# Autodesk Inventor assembly: Servo 250 W
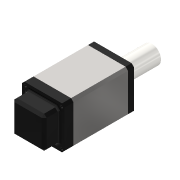
[picture p0: Inventor's stored thumbnail of the model, 180x180]
Saved by Autodesk Inventor 2020.3 (Build 243373010, 373A)
## iProperties
Created: 2021-04-26
Part Number: Servo 250 W
Document SubType Name: Assembly
Designer: marti
Author: marti
## Documents named in this file (8)
- C:\Users\marti\Documents\Inventor\RobotManipulateArm\17.4.2021 - Complete new IDEA\Servo\Servo 250 W.iam
- C:\Users\marti\Documents\Inventor\RobotManipulateArm\17.4.2021 - Complete new IDEA\Servo\Back cover for servo motor 250 W.ipt
- C:\Users\marti\Documents\Inventor\RobotManipulateArm\17.4.2021 - Complete new IDEA\Servo\Cover for servo motor 250 W.ipt
- C:\Users\marti\Documents\Inventor\RobotManipulateArm\17.4.2021 - Complete new IDEA\Servo\Front cover for servo motor 250 W.ipt
- C:\Users\marti\Documents\Inventor\RobotManipulateArm\17.4.2021 - Complete new IDEA\Servo\Stator for 250W servo.iam
- C:\Users\marti\Documents\Inventor\RobotManipulateArm\17.4.2021 - Complete new IDEA\Servo\Rotor assembly for 250W servo.iam
- C:\Users\marti\Documents\Inventor\RobotManipulateArm\17.4.2021 - Complete new IDEA\Servo\Shaft2.ipt
- C:\Users\marti\Documents\Inventor\Content Center Files\R2020\en-US\CSN 02 2562  A\CSN 02 2562 - 5x5x14.ipt
## Components (8 placed, 7 different names)
1. Back cover for servo motor 250 W:1 — Mate:25, Mate:26, Mate:27
2. Cover for servo motor 250 W:1 — Mate:1, Flush:1, Mate:2, Mate:3, Mate:18, Mate:19, Mate:20, Mate:25, Mate:26, Mate:27
3. Front cover for servo motor 250 W:1 — Mate:18, Mate:19, Mate:20
4. Stator for 250W servo:1 [sub-assembly] — Mate:1, Flush:1, Mate:4, Rotation:1, Angle:1, Flush:2
5. Rotor assembly for 250W servo:1 [sub-assembly] — Mate:4, Rotation:1, Angle:1, Flush:2, Mate:21, Mate:22, Mate:23, Mate:24
6. Shaft:1 — Mate:8, Mate:9, Mate:10, Mate:11, Mate:12, Mate:13, Mate:21
7. CSN 02 2562 A 5x5x14:2 — Mate:8, Mate:9, Mate:10, Mate:22, Mate:23
8. CSN 02 2562 A 5x5x14:1 — Mate:11, Mate:12, Mate:13, Mate:24
## Relationships (24: Mate 20, Flush 2, RelateRotation 1, Angle 1)
- Mate:1: Cover for servo motor 250 W:1 ↔ Stator for 250W servo:1
- Flush:1: Cover for servo motor 250 W:1 ↔ Stator for 250W servo:1
- Mate:2: Cover for servo motor 250 W:1
- Mate:3: Cover for servo motor 250 W:1
- Mate:4: Stator for 250W servo:1 ↔ Rotor assembly for 250W servo:1
- Rotation:1 [RelateRotation] (0.2727 ul): Stator for 250W servo:1 ↔ Rotor assembly for 250W servo:1
- Angle:1 (0 deg): Stator for 250W servo:1 ↔ Rotor assembly for 250W servo:1
- Flush:2: Stator for 250W servo:1 ↔ Rotor assembly for 250W servo:1
- Mate:8: Shaft:1 ↔ CSN 02 2562 A 5x5x14:2
- Mate:9: Shaft:1 ↔ CSN 02 2562 A 5x5x14:2
- Mate:10: Shaft:1 ↔ CSN 02 2562 A 5x5x14:2
- Mate:11: Shaft:1 ↔ CSN 02 2562 A 5x5x14:1
- Mate:12: Shaft:1 ↔ CSN 02 2562 A 5x5x14:1
- Mate:13: Shaft:1 ↔ CSN 02 2562 A 5x5x14:1
- Mate:18: Cover for servo motor 250 W:1 ↔ Front cover for servo motor 250 W:1
- Mate:19: Cover for servo motor 250 W:1 ↔ Front cover for servo motor 250 W:1
- Mate:20: Cover for servo motor 250 W:1 ↔ Front cover for servo motor 250 W:1
- Mate:21: Rotor assembly for 250W servo:1 ↔ Shaft:1
- Mate:22: Rotor assembly for 250W servo:1 ↔ CSN 02 2562 A 5x5x14:2
- Mate:23: Rotor assembly for 250W servo:1 ↔ CSN 02 2562 A 5x5x14:2
- Mate:24 (-2.5 mm): Rotor assembly for 250W servo:1 ↔ CSN 02 2562 A 5x5x14:1
- Mate:25: Back cover for servo motor 250 W:1 ↔ Cover for servo motor 250 W:1
- Mate:26: Back cover for servo motor 250 W:1 ↔ Cover for servo motor 250 W:1
- Mate:27: Back cover for servo motor 250 W:1 ↔ Cover for servo motor 250 W:1
